# Autodesk Inventor assembly: 托带轮合
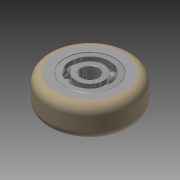
[picture p0: Inventor's stored thumbnail of the model, 180x180]
Saved by Autodesk Inventor 2015 (Build 190159000, 159)
## iProperties
Created: 2017-05-11
Part Number: 托带轮合
Document SubType Name: Assembly
Designer: Administrator
Author: Administrator
## Documents named in this file (3)
- C:\Users\Administrator\Desktop\毕设改\托带轮合.iam
- C:\Users\Administrator\Desktop\毕设改\托带轮.ipt
- C:\Users\Administrator\Desktop\毕设改\托带轮轴承.iam
## Components (3 placed, 2 different names)
1. 托带轮:1 — 插入:1, 插入:2
2. 托带轮轴承:1 [sub-assembly] — 插入:1
3. 托带轮轴承:2 [sub-assembly] — 插入:2
## Relationships (2: Insert 2)
- 插入:1 [Insert]: 托带轮:1 ↔ 托带轮轴承:1
- 插入:2 [Insert]: 托带轮:1 ↔ 托带轮轴承:2
